# Autodesk Inventor assembly: robot
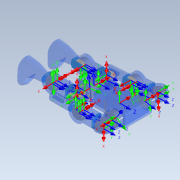
[picture p0: Inventor's stored thumbnail of the model, 180x180]
Saved by Autodesk Inventor 2020 (Build 240168000, 168)
## iProperties
Created: 2021-03-27
Part Number: robot
Document SubType Name: Assembly
Designer: DELL
Author: DELL
## Documents named in this file (9)
- F:\SoftRobot2.0\FlexipodHardware2.0\FlexipodHardware\Flexipod2.0\simulation\pybullete\robot.iam
- F:\SoftRobot2.0\FlexipodHardware2.0\FlexipodHardware\Flexipod2.0\simulation\pybullete\motor.ipt
- F:\SoftRobot2.0\FlexipodHardware2.0\FlexipodHardware\Flexipod2.0\simulation\pybullete\hip.ipt
- F:\SoftRobot2.0\FlexipodHardware2.0\FlexipodHardware\Flexipod2.0\simulation\pybullete\thigh_connector.ipt
- F:\SoftRobot2.0\FlexipodHardware2.0\FlexipodHardware\Flexipod2.0\simulation\pybullete\thigh.ipt
- F:\SoftRobot2.0\FlexipodHardware2.0\FlexipodHardware\Flexipod2.0\simulation\pybullete\shank_connector.ipt
- F:\SoftRobot2.0\FlexipodHardware2.0\FlexipodHardware\Flexipod2.0\simulation\pybullete\shank.ipt
- F:\SoftRobot2.0\FlexipodHardware2.0\FlexipodHardware\Flexipod2.0\simulation\pybullete\body_stand_up_2.ipt
- F:\SoftRobot2.0\FlexipodHardware2.0\FlexipodHardware\Flexipod2.0\simulation\pybullete\shank_back.ipt
## Components (33 placed, 8 different names)
1. body_stand_up_2:1 — Flush:14, Flush:15, Flush:16, Mate:84, Mate:85, Mate:86, Mate:88, Mate:89, Mate:90, Mate:91, Mate:92, Mate:93, Mate:94
2. motor:1 — Mate:42, Mate:89, Mate:90
3. motor:2 — Mate:9, Mate:92, Mate:93
4. motor:3 — Mate:39, Mate:40, Mate:84, Mate:85
5. motor:4 — Mate:11, Mate:86, Mate:87, Mate:88
6. hip:1 — Mate:9, Mate:23, Mate:24, Mate:30, Mate:94
7. hip:2 — Mate:11, Mate:19, Mate:20, Mate:26, Mate:87
8. motor:5 — Mate:31, Mate:43, Mate:44, Mate:46
9. motor:6 — Mate:23, Mate:24, Mate:29
10. motor:7 — Mate:27, Mate:47, Mate:48, Mate:49
11. motor:8 — Mate:19, Mate:20, Mate:25
12. thigh_connector:1 — Mate:29, Mate:30, Mate:34, Flush:5, Flush:9, Mate:71
13. thigh_connector:2 — Mate:31, Mate:33, Flush:4, Mate:37, Mate:44, Mate:45
14. thigh_connector:3 — Mate:27, Mate:36, Flush:7, Mate:38, Mate:49, Mate:50, Mate:77
15. thigh_connector:4 — Mate:25, Mate:26, Mate:35, Flush:6, Flush:8
16. thigh:1 — Mate:34, Flush:5, Flush:9, Mate:55, Mate:56, Angle:18, Mate:60
17. thigh:2 — Mate:36, Flush:7, Mate:38, Mate:51, Mate:52, Angle:20, Mate:62, Angle:23, Mate:81
18. thigh:3 — Mate:33, Flush:4, Mate:37, Mate:57, Mate:58, Angle:17, Mate:66
19. thigh:4 — Mate:35, Flush:6, Flush:8, Mate:53, Mate:54, Angle:19, Mate:64, Flush:17
20. hip:3 — Mate:42, Mate:43, Mate:45, Mate:46, Mate:91
21. hip:4 — Mate:39, Mate:40, Mate:47, Mate:48, Mate:50
22. motor:9 — Mate:51, Mate:52, Angle:20, Mate:61, Flush:13, Mate:78
23. motor:10 — Mate:55, Mate:56, Angle:18, Mate:59, Flush:10, Mate:72
24. motor:11 — Mate:57, Mate:58, Angle:17, Mate:65, Flush:11
25. motor:12 — Mate:53, Mate:54, Angle:19, Mate:63, Flush:12
26. shank_connector:1 — Mate:59, Mate:60, Flush:10, Mate:70, Mate:73
27. shank_connector:2 — Mate:61, Mate:62, Flush:13, Mate:82
28. shank_connector:3 — Mate:65, Mate:66, Flush:11, Mate:69, Mate:76
29. shank_connector:4 — Mate:63, Mate:64, Flush:12, Mate:83
30. shank:2 — Mate:70, Mate:73
31. shank:3 — Mate:69, Mate:76
32. shank_back:1 — Mate:81, Mate:82
33. shank_back:2 — Flush:17, Mate:83
## Relationships (86: Mate 67, Flush 14, Angle 5)
- Mate:9: motor:2 ↔ hip:1
- Mate:11: motor:4 ↔ hip:2
- Mate:19: hip:2 ↔ motor:8
- Mate:20: hip:2 ↔ motor:8
- Mate:23: hip:1 ↔ motor:6
- Mate:24: hip:1 ↔ motor:6
- Mate:25: motor:8 ↔ thigh_connector:4
- Mate:26: hip:2 ↔ thigh_connector:4
- Mate:27: motor:7 ↔ thigh_connector:3
- Mate:29: motor:6 ↔ thigh_connector:1
- Mate:30: hip:1 ↔ thigh_connector:1
- Mate:31: motor:5 ↔ thigh_connector:2
- Mate:33: thigh_connector:2 ↔ thigh:3
- Mate:34: thigh_connector:1 ↔ thigh:1
- Mate:35: thigh_connector:4 ↔ thigh:4
- Mate:36: thigh_connector:3 ↔ thigh:2
- Flush:4: thigh_connector:2 ↔ thigh:3
- Flush:5: thigh_connector:1 ↔ thigh:1
- Flush:6: thigh_connector:4 ↔ thigh:4
- Flush:7: thigh_connector:3 ↔ thigh:2
- Flush:8: thigh_connector:4 ↔ thigh:4
- Mate:37: thigh_connector:2 ↔ thigh:3
- Mate:38: thigh_connector:3 ↔ thigh:2
- Flush:9: thigh_connector:1 ↔ thigh:1
- Mate:39: motor:3 ↔ hip:4
- Mate:40: motor:3 ↔ hip:4
- Mate:42: motor:1 ↔ hip:3
- Mate:43: motor:5 ↔ hip:3
- Mate:44: motor:5 ↔ thigh_connector:2
- Mate:45: thigh_connector:2 ↔ hip:3
- Mate:46: motor:5 ↔ hip:3
- Mate:47: motor:7 ↔ hip:4
- Mate:48: motor:7 ↔ hip:4
- Mate:49: motor:7 ↔ thigh_connector:3
- Mate:50: thigh_connector:3 ↔ hip:4
- Mate:51: thigh:2 ↔ motor:9
- Mate:52: thigh:2 ↔ motor:9
- Mate:53: thigh:4 ↔ motor:12
- Mate:54: thigh:4 ↔ motor:12
- Mate:55: thigh:1 ↔ motor:10
- Mate:56: thigh:1 ↔ motor:10
- Mate:57: thigh:3 ↔ motor:11
- Mate:58: thigh:3 ↔ motor:11
- Angle:17 (0 deg): thigh:3 ↔ motor:11
- Angle:18 (0 deg): thigh:1 ↔ motor:10
- Angle:19 (0 deg): thigh:4 ↔ motor:12
- Angle:20 (0 deg): thigh:2 ↔ motor:9
- Mate:59: motor:10 ↔ shank_connector:1
- Mate:60: thigh:1 ↔ shank_connector:1
- Mate:61: motor:9 ↔ shank_connector:2
- Mate:62: thigh:2 ↔ shank_connector:2
- Mate:63: motor:12 ↔ shank_connector:4
- Mate:64: thigh:4 ↔ shank_connector:4
- Mate:65: motor:11 ↔ shank_connector:3
- Mate:66: thigh:3 ↔ shank_connector:3
- Flush:10: motor:10 ↔ shank_connector:1
- Flush:11: motor:11 ↔ shank_connector:3
- Flush:12: motor:12 ↔ shank_connector:4
- Flush:13: motor:9 ↔ shank_connector:2
- Mate:69: shank_connector:3 ↔ shank:3
- Mate:70: shank_connector:1 ↔ shank:2
- Mate:71: thigh_connector:1
- Mate:72: motor:10
- Mate:73: shank_connector:1 ↔ shank:2
- Mate:76: shank_connector:3 ↔ shank:3
- Mate:77: thigh_connector:3
- Angle:23 (0 deg): thigh:2
- Mate:78: motor:9
- Flush:14: body_stand_up_2:1
- Flush:15: body_stand_up_2:1
- Flush:16: body_stand_up_2:1
- Mate:81: thigh:2 ↔ shank_back:1
- Flush:17: thigh:4 ↔ shank_back:2
- Mate:82: shank_connector:2 ↔ shank_back:1
- Mate:83: shank_connector:4 ↔ shank_back:2
- Mate:84: body_stand_up_2:1 ↔ motor:3
- Mate:85: body_stand_up_2:1 ↔ motor:3
- Mate:86: body_stand_up_2:1 ↔ motor:4
- Mate:87: motor:4 ↔ hip:2
- Mate:88: body_stand_up_2:1 ↔ motor:4
- Mate:89: body_stand_up_2:1 ↔ motor:1
- Mate:90: body_stand_up_2:1 ↔ motor:1
- Mate:91: body_stand_up_2:1 ↔ hip:3
- Mate:92: body_stand_up_2:1 ↔ motor:2
- Mate:93: body_stand_up_2:1 ↔ motor:2
- Mate:94: body_stand_up_2:1 ↔ hip:1
